# Autodesk Inventor assembly: Timing_Assy
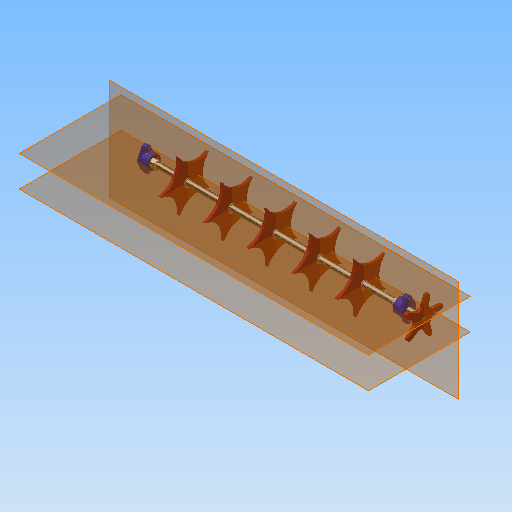
[picture p0: Inventor's stored thumbnail of the model, 512x512]
Saved by Autodesk Inventor 2018.1 (Build 221171000, 171)
## iProperties
Created: 2019-02-11
Part Number: Timing_Assy
Document SubType Name: Assembly
Designer: James
Mass: 92.827 g
Surface Area: 261.339 cm^2
Volume: 33.0472 cm^3
Density: 2.80892 g/cm^3
Author: James
## Documents named in this file (6)
- C:\Users\admin\Desktop\Ball Sorting Machine\Ball-Sorting-Machine\Prototype CAD\Timing Gate - 40mm\Prototype_Assy_Star Shaft.iam
- C:\Users\admin\Desktop\Ball Sorting Machine\Ball-Sorting-Machine\Prototype CAD\Timing Gate - 40mm\Prototype_Star.ipt
- C:\Users\admin\Desktop\Ball Sorting Machine\Ball-Sorting-Machine\Prototype CAD\Timing Gate - 40mm\BS 3673 - 6mm External Circlip.ipt
- C:\Users\admin\Desktop\Ball Sorting Machine\Ball-Sorting-Machine\Prototype CAD\Timing Gate - 40mm\Prototype_Star Shaft.ipt
- C:\Users\admin\Desktop\Ball Sorting Machine\Ball-Sorting-Machine\Prototype CAD\Timing Gate - 40mm\SAFL212 Oval 2 Bolt Flanged Unit.ipt
- C:\Users\admin\Desktop\Ball Sorting Machine\Ball-Sorting-Machine\Prototype CAD\Selection Sort - 40mm\Prototype_Gear 1.ipt
## Components (16 placed, 5 different names)
1. Prototype_Star Shaft:1 — Mate:4, Flush:6, Flush:14, Flush:15, Mate:49, Mate:50, Angle:3, Mate:61, Mate:62, Mate:63, Mate:66, Flush:28, Mate:68, Mate:69, Mate:70
2. SAFL212 Oval 2 Bolt Flanged Unit:1 — Mate:61, Flush:24, Angle:4, Mate:65
3. SAFL212 Oval 2 Bolt Flanged Unit:2 — Mate:62, Flush:24, Mate:64, Mate:67
4. BS 3673 - 6mm External Circlip:16 — Mate:65, Mate:66, Flush:25, Mate:68
5. BS 3673 - 6mm External Circlip:17 — Mate:63, Mate:64, Flush:25, Flush:26
6. Prototype_Gear 1:1 — Mate:69, Mate:70, Angle:5
7. BS 3673 - 6mm External Circlip:11 — Mate:49, Mate:50, Angle:3, Flush:26
8. Prototype_Star:1 — Mate:4, Flush:28, Angle:5
9. BS 3673 - 6mm External Circlip:12
10. Prototype_Star:2
11. BS 3673 - 6mm External Circlip:13
12. Prototype_Star:3
13. BS 3673 - 6mm External Circlip:14
14. Prototype_Star:4
15. BS 3673 - 6mm External Circlip:15
16. Prototype_Star:5
## Component patterns: (5 elements, first: BS 3673 - 6mm External Circlip:11 + Prototype_Star:1)
## Relationships (26: Mate 13, Flush 10, Angle 3)
- Mate:4: Prototype_Star Shaft:1 ↔ Prototype_Star:1
- Flush:6: Prototype_Star Shaft:1
- Flush:11 (-58 mm)
- Flush:12 (-5 mm)
- Flush:13 (30 mm)
- Flush:14: Prototype_Star Shaft:1
- Flush:15: Prototype_Star Shaft:1
- Mate:49: Prototype_Star Shaft:1 ↔ BS 3673 - 6mm External Circlip:11
- Mate:50: Prototype_Star Shaft:1 ↔ BS 3673 - 6mm External Circlip:11
- Angle:3 (0 deg): Prototype_Star Shaft:1 ↔ BS 3673 - 6mm External Circlip:11
- Mate:61: Prototype_Star Shaft:1 ↔ SAFL212 Oval 2 Bolt Flanged Unit:1
- Mate:62: Prototype_Star Shaft:1 ↔ SAFL212 Oval 2 Bolt Flanged Unit:2
- Flush:24: SAFL212 Oval 2 Bolt Flanged Unit:1 ↔ SAFL212 Oval 2 Bolt Flanged Unit:2
- Angle:4 (0 deg): SAFL212 Oval 2 Bolt Flanged Unit:1
- Mate:63: Prototype_Star Shaft:1 ↔ BS 3673 - 6mm External Circlip:17
- Mate:64: SAFL212 Oval 2 Bolt Flanged Unit:2 ↔ BS 3673 - 6mm External Circlip:17
- Mate:65: SAFL212 Oval 2 Bolt Flanged Unit:1 ↔ BS 3673 - 6mm External Circlip:16
- Mate:66: Prototype_Star Shaft:1 ↔ BS 3673 - 6mm External Circlip:16
- Flush:25: BS 3673 - 6mm External Circlip:16 ↔ BS 3673 - 6mm External Circlip:17
- Flush:26: BS 3673 - 6mm External Circlip:17 ↔ BS 3673 - 6mm External Circlip:11
- Mate:67: SAFL212 Oval 2 Bolt Flanged Unit:2
- Flush:28: Prototype_Star Shaft:1 ↔ Prototype_Star:1
- Mate:68: Prototype_Star Shaft:1 ↔ BS 3673 - 6mm External Circlip:16
- Mate:69: Prototype_Star Shaft:1 ↔ Prototype_Gear 1:1
- Mate:70: Prototype_Star Shaft:1 ↔ Prototype_Gear 1:1
- Angle:5 (30 deg): Prototype_Gear 1:1 ↔ Prototype_Star:1
